# Autodesk Inventor assembly: Winch Assembly
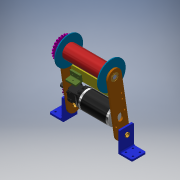
[picture p0: Inventor's stored thumbnail of the model, 180x180]
Saved by Autodesk Inventor 2017 (Build 210142000, 142)
## iProperties
Created: 2017-01-26
Part Number: Winch Assembly
Description: STEP AP214
Document SubType Name: Assembly
Designer: Ben
Sending System: SolidWorks 2015
Preprocessor: SwSTEP 2.0
Title: climb_assy_w_brackets.STEP
Revision Number: ANY
## Documents named in this file (4)
- C:\Users\Ben\Desktop\Projects\2017 Robot\Winch\Winch Assembly.iam
- C:\Users\Ben\Desktop\Projects\2017 Robot\Winch\climber_assembly.iam
- C:\Users\Ben\Desktop\Projects\2017 Robot\Winch\climber_bracket.ipt
- C:\Users\Ben\Desktop\Projects\2017 Robot\Winch\6338K418_OIL-EMBEDDED FLANGED SLEEVE BRNG_6338K418.ipt
## Components (5 placed, 5 different names)
1. climber_assembly_1 [sub-assembly] — Insert:6, Insert:7, Flush:1
2. climber_bracket_2 — Insert:2, Mate:1, Mate:2, Angle:1
3. climber_bracket_3 — Insert:5, Angle:1
4. 6338K418_OIL-EMBEDDED FLANGED SLEEVE BRNG_6338K418_4 — Insert:5, Insert:7
5. 6338K418_OIL-EMBEDDED FLANGED SLEEVE BRNG_6338K418_7 — Insert:2, Insert:6
## Relationships (8: Insert 4, Mate 2, Angle 1, Flush 1)
- Insert:2: climber_bracket_2 ↔ 6338K418_OIL-EMBEDDED FLANGED SLEEVE BRNG_6338K418_7
- Insert:5: climber_bracket_3 ↔ 6338K418_OIL-EMBEDDED FLANGED SLEEVE BRNG_6338K418_4
- Mate:1: climber_bracket_2
- Mate:2 (6.35 mm): climber_bracket_2
- Insert:6 (3.175 mm): climber_assembly_1 ↔ 6338K418_OIL-EMBEDDED FLANGED SLEEVE BRNG_6338K418_7
- Insert:7 (3.175 mm): climber_assembly_1 ↔ 6338K418_OIL-EMBEDDED FLANGED SLEEVE BRNG_6338K418_4
- Angle:1 (0 deg): climber_bracket_2 ↔ climber_bracket_3
- Flush:1: climber_assembly_1
